# Autodesk Inventor assembly: bottom box with container
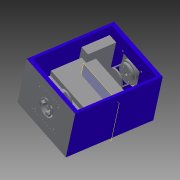
[picture p0: Inventor's stored thumbnail of the model, 180x180]
Saved by Autodesk Inventor 2015 (Build 190159000, 159)
## iProperties
Created: 2014-09-09
Part Number: bottom box with container
Document SubType Name: Assembly
Designer: ericd_000
Author: ericd_000
## Documents named in this file (7)
- C:\Users\ericd_000\Dropbox\GitHub\initial_cad\eric_cad\bottom box with container.iam
- C:\Users\ericd_000\Dropbox\GitHub\initial_cad\eric_cad\bayonet container.ipt
- C:\Users\ericd_000\Dropbox\GitHub\initial_cad\eric_cad\brain box bottom.ipt
- C:\Users\ericd_000\Dropbox\GitHub\initial_cad\eric_cad\bbb brick.ipt
- C:\Users\ericd_000\Dropbox\GitHub\initial_cad\eric_cad\anker20Ah.ipt
- C:\Users\ericd_000\Dropbox\GitHub\initial_cad\eric_cad\nucI5.ipt
- C:\Users\ericd_000\Dropbox\GitHub\initial_cad\eric_cad\tplinkethswitch.ipt
## Components (9 placed, 6 different names)
1. brain box bottom:1 — Rigid:1, Rotational:1, Rotational:2, Mate:1, Mate:2, Mate:3, Mate:4, Mate:5, Mate:7, Mate:8, Mate:9, Mate:11, Mate:13
2. bayonet container:2 — Rigid:1
3. bayonet container:3 — Rotational:1, Mate:4
4. bbb brick:1 — Mate:1, Mate:2
5. bayonet container:4 — Rotational:2, Mate:3, Mate:10
6. anker20Ah:1 — Mate:10, Mate:11, Mate:12
7. anker20Ah:2 — Mate:12, Mate:13
8. nucI5:1 — Mate:7, Mate:9
9. tplinkethswitch:1 — Mate:5, Mate:8
## Relationships (15: Mate 12, RevoluteJoint 2, WeldJoint 1)
- Rigid:1 [WeldJoint]: brain box bottom:1 ↔ bayonet container:2
- Rotational:1 [RevoluteJoint]: brain box bottom:1 ↔ bayonet container:3
- Rotational:2 [RevoluteJoint]: brain box bottom:1 ↔ bayonet container:4
- Mate:1: brain box bottom:1 ↔ bbb brick:1
- Mate:2 (2.54 mm): brain box bottom:1 ↔ bbb brick:1
- Mate:3: brain box bottom:1 ↔ bayonet container:4
- Mate:4: brain box bottom:1 ↔ bayonet container:3
- Mate:5: brain box bottom:1 ↔ tplinkethswitch:1
- Mate:7: brain box bottom:1 ↔ nucI5:1
- Mate:8: brain box bottom:1 ↔ tplinkethswitch:1
- Mate:9: brain box bottom:1 ↔ nucI5:1
- Mate:10: bayonet container:4 ↔ anker20Ah:1
- Mate:11: brain box bottom:1 ↔ anker20Ah:1
- Mate:12 (2.54 mm): anker20Ah:1 ↔ anker20Ah:2
- Mate:13: brain box bottom:1 ↔ anker20Ah:2
